# Autodesk Inventor assembly: ZX10-2-12-S+
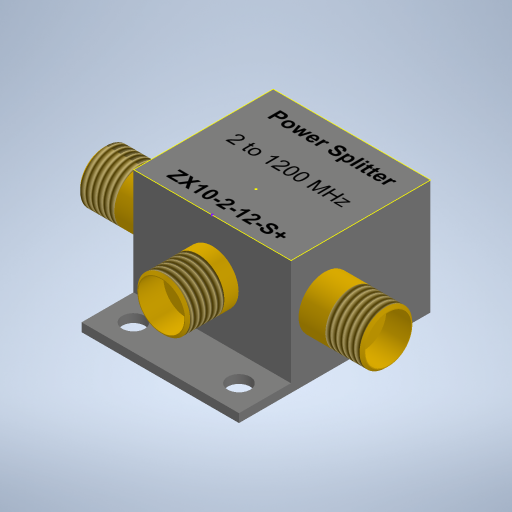
[picture p0: Inventor's stored thumbnail of the model, 512x512]
Saved by Autodesk Inventor 2024 (Build 280153000, 153)
## iProperties
Created: 2023-10-01
Part Number: ZX10-2-12-S+
Document SubType Name: Assembly
Designer: Alexander Pollak
Author: Alexander Pollak
## Documents named in this file (3)
- C:\Users\Alexander Pollak\ownCloud\Inventor\ATA_2019\Shared_Parts\ZX10-2-12-S+\ZX10-2-12-S+.iam
- C:\Users\Alexander Pollak\ownCloud\Inventor\ATA_2019\Shared_Parts\ZX10-2-12-S+\ZX10-2-12-S+.ipt
- C:\Users\Alexander Pollak\ownCloud\Inventor\ATA_2019\Shared_Parts\ZX10-2-12-S+\sma.ipt
## Components (4 placed, 2 different names)
1. ZX10-2-12-S+:1 — Insert:1, Insert:2, Insert:3
2. sma:1 — Insert:3
3. sma:2 — Insert:1
4. sma:3 — Insert:2
## Relationships (3: Insert 3)
- Insert:1 (-1.5 mm): ZX10-2-12-S+:1 ↔ sma:2
- Insert:2: ZX10-2-12-S+:1 ↔ sma:3
- Insert:3: ZX10-2-12-S+:1 ↔ sma:1
